# Autodesk Inventor assembly: FLY MEDIA TUBE ASSY
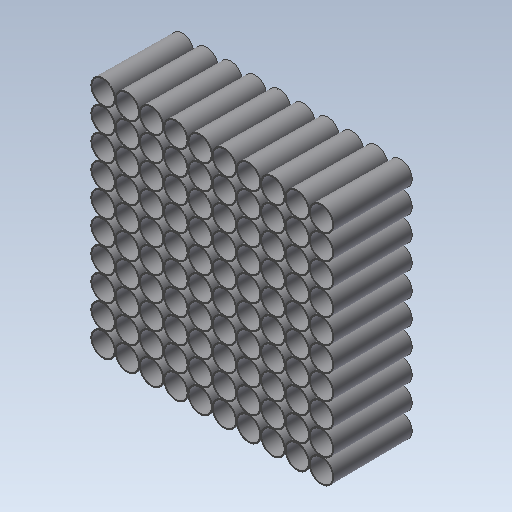
[picture p0: Inventor's stored thumbnail of the model, 512x512]
Saved by Autodesk Inventor 2020.3 (Build 243373000, 373)
## iProperties
RuleStatus: InUse
AfterDocSave0: file://Part Number Cleaner
Created: 2018-09-09
Vendor: HHMI: JRC - ID&F
Document SubType Name: Assembly
Designer: arnoldj
DESIGN DEPARTMENT: HHMI: JRC - ID&F
ALTERED ITEM PART NUMBER: N/A
ALTERED ITEM VENDOR: N/A
ALTERED ITEM DESCRIPTION: N/A
Author: arnoldj
Revision Number: 0
## Documents named in this file (4)
- C:\_WORKSPACE\DATA\PROJECTS\_PROJECTS BY LAB\FLY FACILITY\FLY MEDIA VIAL PLUGGING\FLY MEDIA TUBE ASSY.iam
- C:\_WORKSPACE\DATA\PROJECTS\_PROJECTS BY LAB\FLY FACILITY\FLY MEDIA VIAL PLUGGING\FLY MEDIA TUBE.ipt
- C:\_WORKSPACE\DATA\PROJECTS\_PROJECTS BY LAB\FLY FACILITY\FLY MEDIA VIAL PLUGGING\FLY MEDIA CARDBOARD TRAY.ipt
- C:\_WORKSPACE\DATA\PROJECTS\_PROJECTS BY LAB\FLY FACILITY\FLY MEDIA VIAL PLUGGING\VP 10x10 CAP ASSY.iam
## Components (102 placed, 3 different names)
1. FLY MEDIA CARDBOARD TRAY:1 — Flush:3, Flush:4, Mate:5
2. VP 10x10 CAP ASSY:1 [sub-assembly] — Flush:5, Mate:6, Mate:7
3. FLY MEDIA TUBE:1 — Mate:3, Mate:4
4. FLY MEDIA TUBE:2
5. FLY MEDIA TUBE:3
6. FLY MEDIA TUBE:4
7. FLY MEDIA TUBE:5
8. FLY MEDIA TUBE:6
9. FLY MEDIA TUBE:7
10. FLY MEDIA TUBE:8
11. FLY MEDIA TUBE:9
12. FLY MEDIA TUBE:10 — Mate:5, Flush:5, Mate:7
13. FLY MEDIA TUBE:11
14. FLY MEDIA TUBE:12
15. FLY MEDIA TUBE:13
16. FLY MEDIA TUBE:14
17. FLY MEDIA TUBE:15
18. FLY MEDIA TUBE:16
19. FLY MEDIA TUBE:17
20. FLY MEDIA TUBE:18
21. FLY MEDIA TUBE:19
22. FLY MEDIA TUBE:20
23. FLY MEDIA TUBE:21
24. FLY MEDIA TUBE:22
25. FLY MEDIA TUBE:23
26. FLY MEDIA TUBE:24
27. FLY MEDIA TUBE:25
28. FLY MEDIA TUBE:26
29. FLY MEDIA TUBE:27
30. FLY MEDIA TUBE:28
31. FLY MEDIA TUBE:29
32. FLY MEDIA TUBE:30
33. FLY MEDIA TUBE:31
34. FLY MEDIA TUBE:32
35. FLY MEDIA TUBE:33
36. FLY MEDIA TUBE:34
37. FLY MEDIA TUBE:35
38. FLY MEDIA TUBE:36
39. FLY MEDIA TUBE:37
40. FLY MEDIA TUBE:38
41. FLY MEDIA TUBE:39
42. FLY MEDIA TUBE:40
43. FLY MEDIA TUBE:41
44. FLY MEDIA TUBE:42
45. FLY MEDIA TUBE:43
46. FLY MEDIA TUBE:44
47. FLY MEDIA TUBE:45
48. FLY MEDIA TUBE:46
49. FLY MEDIA TUBE:47
50. FLY MEDIA TUBE:48
51. FLY MEDIA TUBE:49
52. FLY MEDIA TUBE:50
53. FLY MEDIA TUBE:51
54. FLY MEDIA TUBE:52
55. FLY MEDIA TUBE:53
56. FLY MEDIA TUBE:54
57. FLY MEDIA TUBE:55
58. FLY MEDIA TUBE:56
59. FLY MEDIA TUBE:57
60. FLY MEDIA TUBE:58
61. FLY MEDIA TUBE:59
62. FLY MEDIA TUBE:60
63. FLY MEDIA TUBE:61
64. FLY MEDIA TUBE:62
65. FLY MEDIA TUBE:63
66. FLY MEDIA TUBE:64
67. FLY MEDIA TUBE:65
68. FLY MEDIA TUBE:66
69. FLY MEDIA TUBE:67
70. FLY MEDIA TUBE:68
71. FLY MEDIA TUBE:69
72. FLY MEDIA TUBE:70
73. FLY MEDIA TUBE:71
74. FLY MEDIA TUBE:72
75. FLY MEDIA TUBE:73
76. FLY MEDIA TUBE:74
77. FLY MEDIA TUBE:75
78. FLY MEDIA TUBE:76
79. FLY MEDIA TUBE:77
80. FLY MEDIA TUBE:78
81. FLY MEDIA TUBE:79
82. FLY MEDIA TUBE:80
83. FLY MEDIA TUBE:81
84. FLY MEDIA TUBE:82
85. FLY MEDIA TUBE:83
86. FLY MEDIA TUBE:84
87. FLY MEDIA TUBE:85
88. FLY MEDIA TUBE:86
89. FLY MEDIA TUBE:87
90. FLY MEDIA TUBE:88
91. FLY MEDIA TUBE:89
92. FLY MEDIA TUBE:90
93. FLY MEDIA TUBE:91
94. FLY MEDIA TUBE:92
95. FLY MEDIA TUBE:93
96. FLY MEDIA TUBE:94
97. FLY MEDIA TUBE:95
98. FLY MEDIA TUBE:96
99. FLY MEDIA TUBE:97
100. FLY MEDIA TUBE:98
101. FLY MEDIA TUBE:99
102. FLY MEDIA TUBE:100 — Mate:6
## Component patterns: (100 elements, first: FLY MEDIA TUBE:1)
## Relationships (12: Mate 7, Flush 5)
- Flush:1 (129.159 mm)
- Flush:2 (-129.159 mm)
- Mate:1
- Mate:2
- Mate:3: FLY MEDIA TUBE:1
- Mate:4: FLY MEDIA TUBE:1
- Flush:3: FLY MEDIA CARDBOARD TRAY:1
- Flush:4: FLY MEDIA CARDBOARD TRAY:1
- Mate:5: FLY MEDIA CARDBOARD TRAY:1 ↔ FLY MEDIA TUBE:10
- Flush:5 (-14 mm): VP 10x10 CAP ASSY:1 ↔ FLY MEDIA TUBE:10
- Mate:6: VP 10x10 CAP ASSY:1 ↔ FLY MEDIA TUBE:100
- Mate:7: VP 10x10 CAP ASSY:1 ↔ FLY MEDIA TUBE:10
